# Autodesk Inventor assembly: project2_assembly
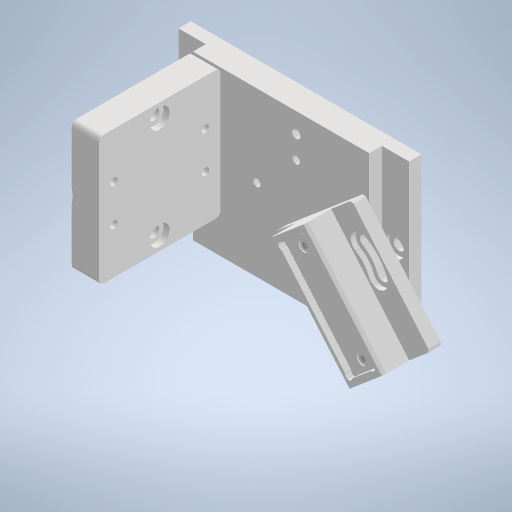
[picture p0: Inventor's stored thumbnail of the model, 512x512]
Saved by Autodesk Inventor 2024.2 (Build 282272000, 272)
## iProperties
Created: 2024-02-21
Part Number: project2_assembly
Document SubType Name: Assembly
Designer: fabig
Author: fabig
## Documents named in this file (4)
- C:\Users\fabig\OneDrive\Documents\GitHub\Git Scheme testing\Parent-folder-table-assembly-\Subproject assemblies\project2-assembly\project2_assembly.iam
- C:\Users\fabig\OneDrive\Documents\GitHub\Git Scheme testing\Parent-folder-table-assembly-\Subproject assemblies\project2-assembly\pegboard-maker-adapter\brimrose\ADAPTER_AOM-brimrose\ADAPTER_AOM-brimrose.ipt
- C:\Users\fabig\OneDrive\Documents\GitHub\Git Scheme testing\Parent-folder-table-assembly-\Subproject assemblies\project2-assembly\pegboard-maker-adapter\intraaction\ADAPTER_AOM-IntraAction\ADAPTER_AOM-IntraAction.ipt
- C:\Users\fabig\OneDrive\Documents\GitHub\Git Scheme testing\Parent-folder-table-assembly-\Subproject assemblies\project2-assembly\pegboard-maker-adapter\qubig\ADAPTER_EOM2.1GHz_new\ADAPTER_EOM2.1GHz_new.ipt
## Components (3 placed, 3 different names)
1. ADAPTER_AOM-brimrose:1 — Mate:1, Mate:2
2. ADAPTER_AOM-IntraAction:1 — Mate:1, Mate:2, Flush:1, Flush:2, Flush:3, Mate:3, Flush:4, Flush:5
3. ADAPTER_EOM2.1GHz_new:1 — Mate:3, Flush:4, Flush:5
## Relationships (8: Flush 5, Mate 3)
- Mate:1: ADAPTER_AOM-brimrose:1 ↔ ADAPTER_AOM-IntraAction:1
- Mate:2: ADAPTER_AOM-brimrose:1 ↔ ADAPTER_AOM-IntraAction:1
- Flush:1: ADAPTER_AOM-IntraAction:1
- Flush:2: ADAPTER_AOM-IntraAction:1
- Flush:3: ADAPTER_AOM-IntraAction:1
- Mate:3: ADAPTER_AOM-IntraAction:1 ↔ ADAPTER_EOM2.1GHz_new:1
- Flush:4: ADAPTER_AOM-IntraAction:1 ↔ ADAPTER_EOM2.1GHz_new:1
- Flush:5: ADAPTER_AOM-IntraAction:1 ↔ ADAPTER_EOM2.1GHz_new:1
